# Autodesk Inventor assembly: left_gripper_cup_with_base
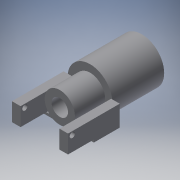
[picture p0: Inventor's stored thumbnail of the model, 180x180]
Saved by Autodesk Inventor 2016 (Build 200138000, 138)
## iProperties
Created: 2016-06-09
Part Number: left_gripper_cup_with_base
Material: 一般
Document SubType Name: Assembly
Designer: Shun Hasegawa
Author: Shun Hasegawa
## Documents named in this file (4)
- C:\Shun\AmazonPickingChallenge\test3\left\left_gripper_cup_with_base.iam
- C:\Shun\AmazonPickingChallenge\test3\left\vacuum_cup_base.ipt
- C:\Shun\AmazonPickingChallenge\test3\vacuum_inlet.ipt
- C:\Shun\AmazonPickingChallenge\test3\vacuum_pad.ipt
## Components (3 placed, 3 different names)
1. vacuum_cup_base:1 — メイト:1, 正接:1, 正接:2, メイト:4, 角度:1
2. vacuum_inlet:1 — メイト:2, メイト:3, 正接:1, 正接:2, メイト:5
3. vacuum_pad:1 — メイト:2, メイト:3, メイト:4
## Relationships (8: Mate 5, Tangent 2, Angle 1)
- メイト:1 [Mate]: vacuum_cup_base:1
- メイト:2 [Mate]: vacuum_inlet:1 ↔ vacuum_pad:1
- メイト:3 [Mate]: vacuum_inlet:1 ↔ vacuum_pad:1
- 正接:1 [Tangent]: vacuum_cup_base:1 ↔ vacuum_inlet:1
- 正接:2 [Tangent] (3 mm): vacuum_cup_base:1 ↔ vacuum_inlet:1
- メイト:4 [Mate]: vacuum_cup_base:1 ↔ vacuum_pad:1
- メイト:5 [Mate]: vacuum_inlet:1
- 角度:1 [Angle] (0 deg): vacuum_cup_base:1
